# Autodesk Inventor assembly: TR2 Arm
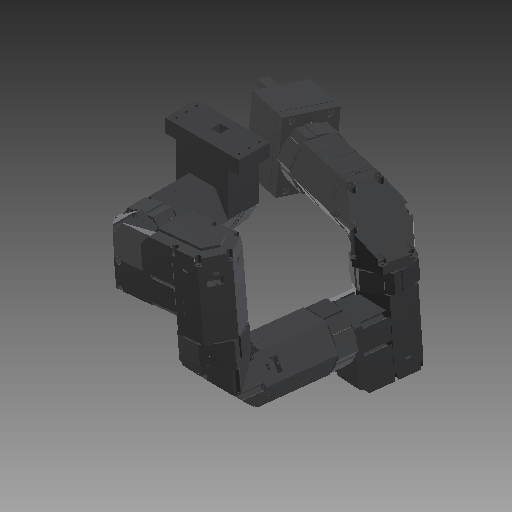
[picture p0: Inventor's stored thumbnail of the model, 512x512]
Saved by Autodesk Inventor 2017 (Build 210142000, 142)
## iProperties
Created: 2018-10-11
Part Number: TR2 Arm
Document SubType Name: Assembly
Designer: Zach
Author: Zach
## Documents named in this file (7)
- C:\Users\Dell\Documents\GitHub\tr2\Arm\Arm.iam
- C:\Users\Dell\Documents\GitHub\tr2\Arm Actuator\Arm Actuator.iam
- C:\Users\Dell\Documents\GitHub\tr2\Gripper\Gripper.iam
- C:\Users\Dell\Documents\GitHub\tr2\Arm\TARM09b.ipt
- C:\Users\Dell\Documents\GitHub\tr2\Arm\TARM01b.ipt
- C:\Users\Dell\Documents\GitHub\tr2\Arm\TARM02b.ipt
- C:\Users\Dell\Documents\GitHub\tr2\Arm\TARM14.ipt
## Components (12 placed, 6 different names)
1. TARM01b:1 — Mate:181, Mate:182, Mate:183
2. Arm Actuator:1 [sub-assembly] — Mate:181, Mate:182, Mate:183, Mate:184, Mate:185
3. Arm Actuator:2 [sub-assembly] — Mate:173, Mate:174, Mate:175, Mate:209, Mate:219
4. Arm Actuator:3 [sub-assembly] — Mate:176, Mate:177, Mate:210, Mate:211, Mate:212
5. Arm Actuator:4 [sub-assembly] — Mate:178, Mate:179, Mate:180, Mate:215, Mate:220
6. Arm Actuator:5 [sub-assembly] — Mate:189, Mate:206, Mate:216, Mate:217, Mate:218
7. Gripper:1 [sub-assembly] — Mate:189, Mate:206
8. TARM09b:1 — Mate:173, Mate:174, Mate:175, Mate:186, Mate:187, Mate:188
9. TARM09b:2 — Mate:176, Mate:177, Mate:178, Mate:179, Mate:180
10. TARM02b:1 — Mate:184, Mate:185, Mate:186, Mate:187, Mate:188
11. TARM14:1 — Mate:209, Mate:210, Mate:211, Mate:212, Mate:219
12. TARM14:2 — Mate:215, Mate:216, Mate:217, Mate:218, Mate:220
## Relationships (28: Mate 28)
- Mate:173: Arm Actuator:2 ↔ TARM09b:1
- Mate:174: Arm Actuator:2 ↔ TARM09b:1
- Mate:175: Arm Actuator:2 ↔ TARM09b:1
- Mate:176: Arm Actuator:3 ↔ TARM09b:2
- Mate:177: Arm Actuator:3 ↔ TARM09b:2
- Mate:178: Arm Actuator:4 ↔ TARM09b:2
- Mate:179: Arm Actuator:4 ↔ TARM09b:2
- Mate:180: Arm Actuator:4 ↔ TARM09b:2
- Mate:181: TARM01b:1 ↔ Arm Actuator:1
- Mate:182: TARM01b:1 ↔ Arm Actuator:1
- Mate:183: TARM01b:1 ↔ Arm Actuator:1
- Mate:184: Arm Actuator:1 ↔ TARM02b:1
- Mate:185: Arm Actuator:1 ↔ TARM02b:1
- Mate:186: TARM09b:1 ↔ TARM02b:1
- Mate:187: TARM09b:1 ↔ TARM02b:1
- Mate:188: TARM09b:1 ↔ TARM02b:1
- Mate:189: Arm Actuator:5 ↔ Gripper:1
- Mate:206: Arm Actuator:5 ↔ Gripper:1
- Mate:209: Arm Actuator:2 ↔ TARM14:1
- Mate:210: Arm Actuator:3 ↔ TARM14:1
- Mate:211: Arm Actuator:3 ↔ TARM14:1
- Mate:212: Arm Actuator:3 ↔ TARM14:1
- Mate:215: Arm Actuator:4 ↔ TARM14:2
- Mate:216: Arm Actuator:5 ↔ TARM14:2
- Mate:217: Arm Actuator:5 ↔ TARM14:2
- Mate:218: Arm Actuator:5 ↔ TARM14:2
- Mate:219: Arm Actuator:2 ↔ TARM14:1
- Mate:220: Arm Actuator:4 ↔ TARM14:2
